# Autodesk Inventor assembly: 205 assembly
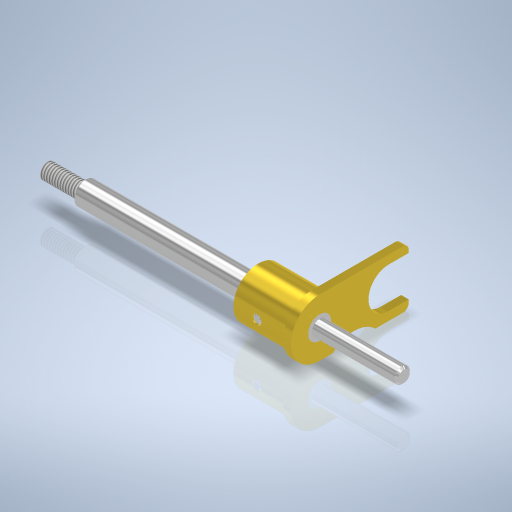
[picture p0: Inventor's stored thumbnail of the model, 512x512]
Saved by Autodesk Inventor 2024 (Build 280153000, 153)
## iProperties
Created: 2024-07-12
Part Number: 205 assembly
Document SubType Name: Assembly
Designer: ffogue
Author: ffogue
## Documents named in this file (5)
- C:\Users\ffogue\OneDrive - MuM - OM\Dokumente\Inventor\GearBox\205 assembly.iam
- C:\Users\ffogue\OneDrive - MuM - OM\Dokumente\Inventor\GearBox\205 part 2.ipt
- C:\Users\ffogue\OneDrive - MuM - OM\Dokumente\Inventor\GearBox\205 part 1.ipt
- C:\Users\ffogue\OneDrive - MuM - OM\Dokumente\Inventor\GearBox\205 part 3.ipt
- C:\Users\ffogue\OneDrive - MuM - OM\Dokumente\Inventor\GearBox\205Bolt.ipt
## Components (4 placed, 4 different names)
1. 205 part 2:1 — Einfügen:1, Passend:1, Zylindrisch:1
2. 205 part 1:1 — Passend:1, Fluchtend:1
3. 205 part 3:1 — Einfügen:1, Fluchtend:1
4. 205Bolt:1 — Zylindrisch:1
## Relationships (4: Insert 1, Mate 1, Flush 1, CylindricalJoint 1)
- Einfügen:1 [Insert]: 205 part 2:1 ↔ 205 part 3:1
- Passend:1 [Mate]: 205 part 2:1 ↔ 205 part 1:1
- Fluchtend:1 [Flush]: 205 part 1:1 ↔ 205 part 3:1
- Zylindrisch:1 [CylindricalJoint]: 205 part 2:1 ↔ 205Bolt:1
